# Autodesk Inventor assembly: EnsembleV1
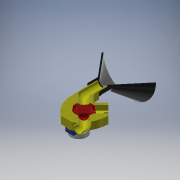
[picture p0: Inventor's stored thumbnail of the model, 180x180]
Saved by Autodesk Inventor 2019 (Build 230136000, 136)
## iProperties
Created: 2020-12-14
Part Number: EnsembleV1
Material: Générique
Document SubType Name: Assembly
Designer: tom.mousset
Author: tom.mousset
## Documents named in this file (5)
- D:\triSmarties\EnsembleV1.iam
- D:\triSmarties\carcasseHaut.ipt
- D:\triSmarties\roue.ipt
- D:\triSmarties\Step - 28BYJ-48.ipt
- D:\triSmarties\entonnoir.ipt
## Components (4 placed, 4 different names)
1. carcasseHaut:1 — Placage:1, Placage:2, Placage:4, Placage:5, Angle:2, Placage:6, Placage:7
2. Step - 28BYJ-48:1 — Placage:1, Placage:2, Angle:1, Angle:2
3. roue:1 — Placage:4, Placage:5, Angle:1
4. entonnoir:1 — Placage:6, Placage:7
## Relationships (8: Mate 6, Angle 2)
- Placage:1 [Mate]: carcasseHaut:1 ↔ Step - 28BYJ-48:1
- Placage:2 [Mate]: carcasseHaut:1 ↔ Step - 28BYJ-48:1
- Placage:4 [Mate]: carcasseHaut:1 ↔ roue:1
- Placage:5 [Mate]: carcasseHaut:1 ↔ roue:1
- Angle:1 (45 deg): Step - 28BYJ-48:1 ↔ roue:1
- Angle:2 (180 deg): carcasseHaut:1 ↔ Step - 28BYJ-48:1
- Placage:6 [Mate]: carcasseHaut:1 ↔ entonnoir:1
- Placage:7 [Mate]: carcasseHaut:1 ↔ entonnoir:1
